# Autodesk Inventor assembly: Cylinder, Bi-directional-empty hole
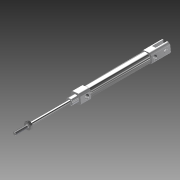
[picture p0: Inventor's stored thumbnail of the model, 180x180]
Saved by Autodesk Inventor 2014 (Build 180170000, 170)
## iProperties
Created: 2011-03-21
Part Number: Cylinder, Bi-directional-empty hole
Document SubType Name: Assembly
Designer: Jordan
Translation Standard: STEP AP203
FileName: Cylinder, Bi-directional.iam
PreProcessor: SolidWorks 2007
PostProcessor: Build: 239, Release: 2011 RTM - Date: Wed 02/17/2010
Sent Units: millimeter
Uncertainty: 1e-05
Author: Jordan
## Documents named in this file (4)
- F:\Inventor\Robotics\Vex parts\Other Parts\Cylinder, Bi-directional-empty hole.iam
- F:\Inventor\Robotics\Vex parts\Other Parts\Cylinder, Bi-directional-Parts\Nut 8-32 Hex.ipt
- F:\Inventor\Robotics\Vex parts\Other Parts\Cylinder, Bi-directional-Parts\Rod.ipt
- F:\Inventor\Robotics\Vex parts\Other Parts\Cylinder, Bi-directional-Parts\Body.ipt
## Components (3 placed, 3 different names)
1. Nut 8-32 Hex:1 — Insert:1
2. Rod:1 — Mate:1, Insert:1
3. Body:1 — Mate:1
## Relationships (2: Mate 1, Insert 1)
- Mate:1: Rod:1 ↔ Body:1
- Insert:1: Nut 8-32 Hex:1 ↔ Rod:1
